# Autodesk Inventor assembly: Montagem_corpo
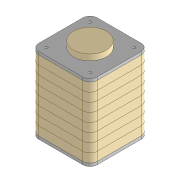
[picture p0: Inventor's stored thumbnail of the model, 180x180]
Saved by Autodesk Inventor 2020 (Build 240168000, 168)
## iProperties
Created: 2022-07-20
Part Number: Montagem_corpo
Document SubType Name: Assembly
Designer: gabri
Author: gabri
## Documents named in this file (7)
- C:\Users\gabri\OneDrive\Área de Trabalho\Calorimetro 2022\Inventor\Montagem_corpo.iam
- C:\Users\gabri\OneDrive\Área de Trabalho\Calorimetro 2022\Inventor\suporte-superior2.ipt
- C:\Users\gabri\OneDrive\Área de Trabalho\Calorimetro 2022\Inventor\suporte-superior.ipt
- C:\Users\gabri\OneDrive\Área de Trabalho\Calorimetro 2022\Inventor\corpo_01a.ipt
- C:\Users\gabri\OneDrive\Área de Trabalho\Calorimetro 2022\Inventor\corpo_01b.ipt
- C:\Users\gabri\OneDrive\Área de Trabalho\Calorimetro 2022\Inventor\tampa.ipt
- C:\Users\gabri\OneDrive\Área de Trabalho\Calorimetro 2022\Inventor\porcaM4.ipt
## Components (15 placed, 6 different names)
1. suporte-superior2:1 — Coincidência:4, Alinhamento:7, Alinhamento:8
2. suporte-superior:1 — Coincidência:1, Alinhamento:1, Alinhamento:2, Coincidência:7, Coincidência:8, Coincidência:9, Coincidência:10, Coincidência:11, Coincidência:12, Coincidência:13, Coincidência:14
3. corpo_01a:1 — Coincidência:1, Alinhamento:1, Alinhamento:2, Coincidência:2, Alinhamento:3, Alinhamento:4
4. tampa:1 — Coincidência:5, Coincidência:6
5. porcaM4:1 — Coincidência:10, Coincidência:13
6. porcaM4:2 — Coincidência:7, Coincidência:11
7. porcaM4:3 — Coincidência:8, Coincidência:12
8. porcaM4:4 — Coincidência:9, Coincidência:14
9. corpo_01b:1 — Coincidência:2, Alinhamento:3, Alinhamento:4
10. corpo_01b:2
11. corpo_01b:3
12. corpo_01b:4 — Coincidência:3, Alinhamento:5, Alinhamento:6
13. corpo_01a:2 — Coincidência:3, Alinhamento:5, Alinhamento:6
14. corpo_01a:3
15. corpo_01a:4 — Coincidência:4, Alinhamento:7, Alinhamento:8, Coincidência:5, Coincidência:6
## Component patterns: (4 elements, first: corpo_01b:1), (3 elements, first: corpo_01a:2)
## Relationships (22: Mate 14, Flush 8)
- Coincidência:1 [Mate]: suporte-superior:1 ↔ corpo_01a:1
- Alinhamento:1 [Flush]: suporte-superior:1 ↔ corpo_01a:1
- Alinhamento:2 [Flush]: suporte-superior:1 ↔ corpo_01a:1
- Coincidência:2 [Mate]: corpo_01a:1 ↔ corpo_01b:1
- Alinhamento:3 [Flush]: corpo_01a:1 ↔ corpo_01b:1
- Alinhamento:4 [Flush]: corpo_01a:1 ↔ corpo_01b:1
- Coincidência:3 [Mate]: corpo_01b:4 ↔ corpo_01a:2
- Alinhamento:5 [Flush]: corpo_01b:4 ↔ corpo_01a:2
- Alinhamento:6 [Flush]: corpo_01b:4 ↔ corpo_01a:2
- Coincidência:4 [Mate]: suporte-superior2:1 ↔ corpo_01a:4
- Alinhamento:7 [Flush]: suporte-superior2:1 ↔ corpo_01a:4
- Alinhamento:8 [Flush]: suporte-superior2:1 ↔ corpo_01a:4
- Coincidência:5 [Mate]: tampa:1 ↔ corpo_01a:4
- Coincidência:6 [Mate]: tampa:1 ↔ corpo_01a:4
- Coincidência:7 [Mate]: suporte-superior:1 ↔ porcaM4:2
- Coincidência:8 [Mate]: suporte-superior:1 ↔ porcaM4:3
- Coincidência:9 [Mate]: suporte-superior:1 ↔ porcaM4:4
- Coincidência:10 [Mate]: suporte-superior:1 ↔ porcaM4:1
- Coincidência:11 [Mate]: suporte-superior:1 ↔ porcaM4:2
- Coincidência:12 [Mate]: suporte-superior:1 ↔ porcaM4:3
- Coincidência:13 [Mate]: suporte-superior:1 ↔ porcaM4:1
- Coincidência:14 [Mate]: suporte-superior:1 ↔ porcaM4:4
